# Autodesk Inventor assembly: RoboCinWheel_simplified
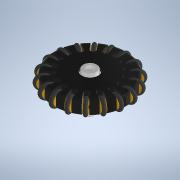
[picture p0: Inventor's stored thumbnail of the model, 180x180]
Saved by Autodesk Inventor 2021 (Build 250183000, 183)
## iProperties
Created: 2022-09-21
Part Number: RoboCinWheel_simplified
Document SubType Name: Assembly
Designer: victo
Author: victo
## Documents named in this file (4)
- C:\Users\victo\Documents\MATLAB\CAD\Inventor\first_floor\Wheel\RoboCinWheel_simplified.iam
- C:\Users\victo\Documents\MATLAB\CAD\Inventor\first_floor\Wheel\wheel_simplified2.ipt
- C:\Users\victo\Documents\MATLAB\CAD\Inventor\first_floor\Wheel\gear_z60_26106000_simplified.ipt
- C:\Users\victo\Documents\MATLAB\CAD\Inventor\first_floor\Wheel\Roller.iam
## Components (20 placed, 3 different names)
1. wheel_simplified2:1 — Mate:1, Mate:2, Mate:3, Mate:4, Mate:5, Mate:6, Mate:7, Mate:8, Mate:9, Mate:10, Mate:11, Mate:12, Mate:13, Mate:14, Mate:15, Mate:16, Mate:17, Mate:18, Mate:19, Mate:20, Mate:21, Mate:22, Mate:23, Mate:24, Mate:25, Mate:26, Mate:27, Mate:28, Mate:29, Mate:30, Mate:31, Mate:32, Mate:33, Mate:34, Mate:35, Mate:36, Mate:37, Mate:38
2. gear_z60_26106000_simplified:1 — Mate:1, Mate:2
3. Roller:1 [sub-assembly] — Mate:3, Mate:4
4. Roller:2 [sub-assembly] — Mate:5, Mate:6
5. Roller:3 [sub-assembly] — Mate:7, Mate:8
6. Roller:4 [sub-assembly] — Mate:9, Mate:10
7. Roller:5 [sub-assembly] — Mate:11, Mate:12
8. Roller:6 [sub-assembly] — Mate:13, Mate:14
9. Roller:7 [sub-assembly] — Mate:15, Mate:16
10. Roller:8 [sub-assembly] — Mate:17, Mate:18
11. Roller:9 [sub-assembly] — Mate:19, Mate:20
12. Roller:10 [sub-assembly] — Mate:21, Mate:22
13. Roller:11 [sub-assembly] — Mate:27, Mate:28
14. Roller:12 [sub-assembly] — Mate:25, Mate:26
15. Roller:13 [sub-assembly] — Mate:23, Mate:24
16. Roller:14 [sub-assembly] — Mate:31, Mate:32
17. Roller:15 [sub-assembly] — Mate:33, Mate:34
18. Roller:16 [sub-assembly] — Mate:29, Mate:30
19. Roller:17 [sub-assembly] — Mate:35, Mate:36
20. Roller:18 [sub-assembly] — Mate:37, Mate:38
## Relationships (38: Mate 38)
- Mate:1: wheel_simplified2:1 ↔ gear_z60_26106000_simplified:1
- Mate:2: wheel_simplified2:1 ↔ gear_z60_26106000_simplified:1
- Mate:3: wheel_simplified2:1 ↔ Roller:1
- Mate:4 (0.15 mm): wheel_simplified2:1 ↔ Roller:1
- Mate:5: wheel_simplified2:1 ↔ Roller:2
- Mate:6 (0.15 mm): wheel_simplified2:1 ↔ Roller:2
- Mate:7: wheel_simplified2:1 ↔ Roller:3
- Mate:8 (0.15 mm): wheel_simplified2:1 ↔ Roller:3
- Mate:9: wheel_simplified2:1 ↔ Roller:4
- Mate:10 (0.15 mm): wheel_simplified2:1 ↔ Roller:4
- Mate:11: wheel_simplified2:1 ↔ Roller:5
- Mate:12 (0.15 mm): wheel_simplified2:1 ↔ Roller:5
- Mate:13: wheel_simplified2:1 ↔ Roller:6
- Mate:14 (0.15 mm): wheel_simplified2:1 ↔ Roller:6
- Mate:15: wheel_simplified2:1 ↔ Roller:7
- Mate:16 (0.15 mm): wheel_simplified2:1 ↔ Roller:7
- Mate:17: wheel_simplified2:1 ↔ Roller:8
- Mate:18 (0.15 mm): wheel_simplified2:1 ↔ Roller:8
- Mate:19: wheel_simplified2:1 ↔ Roller:9
- Mate:20 (0.15 mm): wheel_simplified2:1 ↔ Roller:9
- Mate:21: wheel_simplified2:1 ↔ Roller:10
- Mate:22 (0.15 mm): wheel_simplified2:1 ↔ Roller:10
- Mate:23: wheel_simplified2:1 ↔ Roller:13
- Mate:24 (0.15 mm): wheel_simplified2:1 ↔ Roller:13
- Mate:25: wheel_simplified2:1 ↔ Roller:12
- Mate:26 (0.15 mm): wheel_simplified2:1 ↔ Roller:12
- Mate:27: wheel_simplified2:1 ↔ Roller:11
- Mate:28 (0.15 mm): wheel_simplified2:1 ↔ Roller:11
- Mate:29: wheel_simplified2:1 ↔ Roller:16
- Mate:30 (0.15 mm): wheel_simplified2:1 ↔ Roller:16
- Mate:31: wheel_simplified2:1 ↔ Roller:14
- Mate:32 (0.15 mm): wheel_simplified2:1 ↔ Roller:14
- Mate:33: wheel_simplified2:1 ↔ Roller:15
- Mate:34 (0.15 mm): wheel_simplified2:1 ↔ Roller:15
- Mate:35: wheel_simplified2:1 ↔ Roller:17
- Mate:36 (0.15 mm): wheel_simplified2:1 ↔ Roller:17
- Mate:37: wheel_simplified2:1 ↔ Roller:18
- Mate:38 (0.15 mm): wheel_simplified2:1 ↔ Roller:18
